# Autodesk Inventor assembly: printingLayout
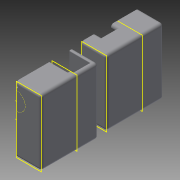
[picture p0: Inventor's stored thumbnail of the model, 180x180]
Saved by Autodesk Inventor 2013 (Build 170138000, 138)
## iProperties
Created: 2012-10-04
Part Number: printingLayout
Document SubType Name: Assembly
Designer: androbin
Author: androbin
## Documents named in this file (3)
- C:\Users\Andrew\Documents\printingLayout.iam
- C:\Users\Andrew\Documents\design.ipt
- C:\Users\Andrew\Documents\design_MIR.ipt
## Components (2 placed, 2 different names)
1. design:2 — Flush:1, Flush:2
2. design_MIR:1 — Flush:1, Flush:2
## Relationships (2: Flush 2)
- Flush:1: design:2 ↔ design_MIR:1
- Flush:2: design:2 ↔ design_MIR:1
